# Autodesk Inventor assembly: Assembly of hinge
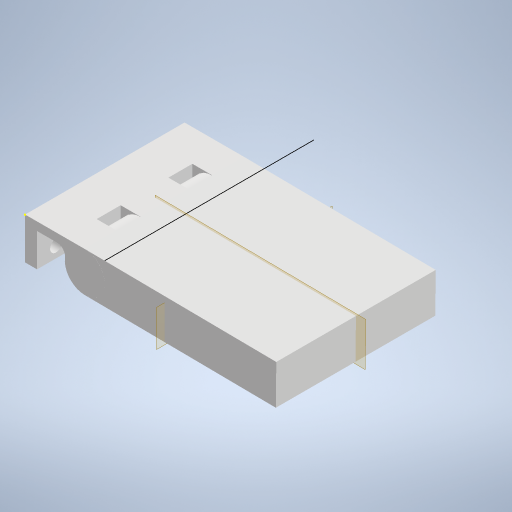
[picture p0: Inventor's stored thumbnail of the model, 512x512]
Saved by Autodesk Inventor 2024.2 (Build 282272000, 272)
## iProperties
Created: 2024-11-15
Part Number: Assembly of hinge
Document SubType Name: Assembly
Designer: Tom
Author: Tom
## Documents named in this file (3)
- C:\Users\Tom\Desktop\UCSF\Preeya UCB\stretchable project\Strain-Sensor-\CAD Files\auto bender part files\Assembly of hinge.iam
- C:\Users\Tom\Desktop\UCSF\Preeya UCB\stretchable project\Strain-Sensor-\CAD Files\auto bender part files\knuckle plate hinge.ipt
- C:\Users\Tom\Desktop\UCSF\Preeya UCB\stretchable project\Strain-Sensor-\CAD Files\auto bender part files\knuckle plate hinge 2.ipt
## Components (2 placed, 2 different names)
1. knuckle plate hinge:1 — Cylindrical:1, Flush:1
2. knuckle plate hinge 2:1 — Cylindrical:1, Flush:1
## Relationships (2: CylindricalJoint 1, Flush 1)
- Cylindrical:1: knuckle plate hinge:1 ↔ knuckle plate hinge 2:1
- Flush:1: knuckle plate hinge:1 ↔ knuckle plate hinge 2:1
